# Autodesk Inventor assembly: Pok Mk3 Demo
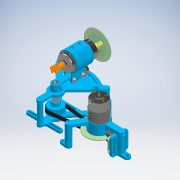
[picture p0: Inventor's stored thumbnail of the model, 180x180]
Saved by Autodesk Inventor 2018.2 (Build 222227000, 227)
## iProperties
Created: 2018-02-12
Part Number: Pok Mk3 Demo
Document SubType Name: Assembly
Designer: Moochster
Author: Moochster
## Documents named in this file (25)
- C:\Users\Moochster\OneDrive\Documents\2018 UBC\ELEC 391\Controller\cad\Pok Mk3 Demo.iam
- C:\Users\Moochster\OneDrive\Documents\2018 UBC\ELEC 391\Controller\cad\Rod 3-8in.ipt
- C:\Users\Moochster\OneDrive\Documents\2018 UBC\ELEC 391\Controller\cad\R1038_ZZ_W Bearing.ipt
- C:\Users\Moochster\OneDrive\Documents\2018 UBC\ELEC 391\Controller\cad\Yaw Platform Top.ipt
- C:\Users\Moochster\OneDrive\Documents\2018 UBC\ELEC 391\Controller\cad\Pok Header Mount.ipt
- C:\Users\Moochster\OneDrive\Documents\2018 UBC\ELEC 391\Controller\cad\JD5B-2655W-R.ipt
- C:\Users\Moochster\OneDrive\Documents\2018 UBC\ELEC 391\Controller\cad\Pok Default Pitch Motor Mount.ipt
- C:\Users\Moochster\OneDrive\Documents\2018 UBC\ELEC 391\Controller\cad\Laser Mount.ipt
- C:\Users\Moochster\Documents\Inventor\Content Center Files\R2018\en-US\AS 1110\AS 1110 - M3 x 20.ipt
- C:\Users\Moochster\Documents\Inventor\Content Center Files\R2018\en-US\AS 1112 (2)\AS 1112 - M3  Type 5.ipt
- C:\Users\Moochster\Documents\Inventor\Content Center Files\R2018\en-US\CNS 5050\CNS 5050 - A - 3.2 8.ipt
- C:\Users\Moochster\Documents\Inventor\Content Center Files\R2018\en-US\ANSI B18.3.1M(1)\ANSI B18.3.1M - M1.6x0.35 x 3(2).ipt
- C:\Users\Moochster\OneDrive\Documents\2018 UBC\ELEC 391\Controller\cad\Pok Mk3 Base.ipt
- C:\Users\Moochster\OneDrive\Documents\2018 UBC\ELEC 391\Controller\cad\Pok Mk3 Support.ipt
- C:\Users\Moochster\OneDrive\Documents\2018 UBC\ELEC 391\Controller\cad\Encoder Wheel (G16).ipt
- C:\Users\Moochster\OneDrive\Documents\2018 UBC\ELEC 391\Controller\cad\Shaft Encoder Adapter.ipt
- C:\Users\Moochster\OneDrive\Documents\2018 UBC\ELEC 391\Controller\cad\GP1A52HRJ00F (Large slot detector).ipt
- C:\Users\Moochster\OneDrive\Documents\2018 UBC\ELEC 391\Controller\cad\GT2 Gear Pinion.ipt
- C:\Users\Moochster\OneDrive\Documents\2018 UBC\ELEC 391\Controller\cad\GT2 Gear Big.ipt
- C:\Users\Moochster\OneDrive\Documents\2018 UBC\ELEC 391\Controller\cad\Pok Mk3 Yaw Motor Support.ipt
- C:\Users\Moochster\OneDrive\Documents\2018 UBC\ELEC 391\Controller\cad\Large Encoder PCB.ipt
- C:\Users\Moochster\OneDrive\Documents\2018 UBC\ELEC 391\Controller\cad\Nylon M3 4mm Spacer.ipt
- C:\Users\Moochster\OneDrive\Documents\2018 UBC\ELEC 391\Controller\cad\Pok Mk3 Yaw Motor Mount Mk2.ipt
- C:\Users\Moochster\OneDrive\Documents\2018 UBC\ELEC 391\Controller\cad\Pok Mk3 Yaw Motor Support Min.ipt
- C:\Users\Moochster\OneDrive\Documents\2018 UBC\ELEC 391\Controller\cad\Belt.ipt
## Components (41 placed, 24 different names)
1. Rod 3-8in:1 — Mate:1, Mate:2, Flush:1, Mate:10, Mate:23, Mate:24, Mate:42, Mate:70, Mate:71
2. R1038_ZZ_W Bearing:1 — Mate:1, Flush:1, Mate:60, Flush:17
3. R1038_ZZ_W Bearing:2 — Mate:2, Mate:5, Flush:2
4. Yaw Platform Top:1 — Mate:5, Flush:2, Mate:11, Angle:1, Insert:16
5. Pok Header Mount:1 — Mate:10, Mate:11, Mate:12, Flush:4, Mate:19, Mate:20, Mate:21, Angle:6, Mate:71
6. R1038_ZZ_W Bearing:3 — Mate:12, Flush:4
7. JD5B-2655W-R:1 — Mate:17, Mate:18, Mate:22, Flush:5, Angle:2, Tangent:1, Tangent:2, Mate:34, Mate:38, Angle:7
8. Laser Mount:1 — Mate:17, Mate:18
9. Pok Default Pitch Motor Mount:1 — Mate:19, Mate:20, Mate:21, Mate:22, Flush:5, Mate:25, Insert:1, Insert:3, Insert:5, Insert:7, Angle:2, Mate:26, Mate:27
10. AS 1110 - Metric M3 x 20:1 — Mate:25, Insert:2
11. AS 1110 - Metric M3 x 20:2 — Insert:6
12. CNS 5050 A - 3.2:4 — Insert:7, Insert:8
13. CNS 5050 A - 3.2:2 — Insert:5, Insert:6
14. CNS 5050 A - 3.2:3 — Insert:3, Insert:4
15. CNS 5050 A - 3.2:1 — Insert:1, Insert:2
16. AS 1112 (2) - Metric M3  Type 5:1 — Insert:8
17. AS 1112 (2) - Metric M3  Type 5:2 — Insert:4
18. Broached Socket Head Cap Screw - Metric M1.6x0.35 x 3:1 — Mate:26, Tangent:1
19. Broached Socket Head Cap Screw - Metric M1.6x0.35 x 3:2 — Mate:27, Tangent:2
20. Pok Mk3 Base:1 — Insert:13, Insert:14, Insert:15, Mate:60, Flush:17, Flush:18, Angle:5, Flush:20, Mate:68, Angle:7
21. Pok Mk3 Support:1 — Insert:13
22. Pok Mk3 Support:2 — Insert:15, Insert:16
23. Pok Mk3 Support:3 — Insert:14
24. JD5B-2655W-R:2 — Mate:32, Mate:41, Mate:44, Mate:53, Mate:55
25. Encoder Wheel (G16):1 — Mate:32, Mate:43, Mate:44, Mate:69
26. Encoder Wheel (G16):2 — Mate:35, Mate:36, Mate:37
27. Shaft Encoder Adapter:1 — Mate:34, Mate:35, Mate:36, Mate:37, Mate:38
28. GP1A52HRJ00F (Large slot detector):3 — Mate:50, Flush:13, Flush:14, Mate:51, Flush:15
29. GP1A52HRJ00F (Large slot detector):4 — Mate:50, Flush:13, Flush:14, Flush:16
30. GT2 Gear Pinion:1 — Mate:41, Mate:43, Flush:10, Mate:67, Mate:69, Rotation:1
31. GT2 Gear Big:1 — Mate:42, Flush:10, Angle:6, Mate:65, Mate:66, Rotation:1, Mate:70
32. Pok Mk3 Yaw Motor Support:4 — Mate:52, Mate:54, Angle:4, Tangent:3, Tangent:4, Mate:62
33. Large Encoder PCB:1 — Mate:51, Flush:15, Flush:16, Mate:52, Insert:9, Insert:10, Insert:11, Insert:12
34. Nylon M3 4mm Spacer:1 — Insert:10, Tangent:4
35. Nylon M3 4mm Spacer:2 — Insert:9
36. Nylon M3 4mm Spacer:3 — Insert:12
37. Nylon M3 4mm Spacer:4 — Insert:11, Tangent:3
38. Pok Mk3 Yaw Motor Mount Mk2:1 — Mate:53, Mate:54, Angle:4, Mate:55, Mate:56, Mate:57, Mate:58, Mate:59, Angle:5, Mate:62, Mate:68
39. Pok Mk3 Yaw Motor Support Min:1 — Mate:56, Mate:58, Mate:64
40. Pok Mk3 Yaw Motor Support Min:2 — Mate:57, Mate:59, Flush:18, Mate:63
41. Belt:1 — Mate:65, Mate:66, Mate:67
## Relationships (87: Mate 48, Insert 16, Flush 12, Angle 6, Tangent 4, RelateRotation 1)
- Mate:1: Rod 3-8in:1 ↔ R1038_ZZ_W Bearing:1
- Mate:2: Rod 3-8in:1 ↔ R1038_ZZ_W Bearing:2
- Flush:1: Rod 3-8in:1 ↔ R1038_ZZ_W Bearing:1
- Mate:5: R1038_ZZ_W Bearing:2 ↔ Yaw Platform Top:1
- Flush:2: R1038_ZZ_W Bearing:2 ↔ Yaw Platform Top:1
- Mate:10: Rod 3-8in:1 ↔ Pok Header Mount:1
- Mate:11 (0.2 mm): Yaw Platform Top:1 ↔ Pok Header Mount:1
- Mate:12: Pok Header Mount:1 ↔ R1038_ZZ_W Bearing:3
- Flush:4 (1 mm): Pok Header Mount:1 ↔ R1038_ZZ_W Bearing:3
- Mate:17: JD5B-2655W-R:1 ↔ Laser Mount:1
- Mate:18 (1 mm): JD5B-2655W-R:1 ↔ Laser Mount:1
- Mate:19: Pok Header Mount:1 ↔ Pok Default Pitch Motor Mount:1
- Mate:20: Pok Header Mount:1 ↔ Pok Default Pitch Motor Mount:1
- Mate:21 (0.1 mm): Pok Header Mount:1 ↔ Pok Default Pitch Motor Mount:1
- Mate:22: JD5B-2655W-R:1 ↔ Pok Default Pitch Motor Mount:1
- Mate:23: Rod 3-8in:1
- Mate:24: Rod 3-8in:1
- Angle:1 (0 deg): Yaw Platform Top:1
- Flush:5 (-10 mm): JD5B-2655W-R:1 ↔ Pok Default Pitch Motor Mount:1
- Mate:25: Pok Default Pitch Motor Mount:1 ↔ AS 1110 - Metric M3 x 20:1
- Insert:1: Pok Default Pitch Motor Mount:1 ↔ CNS 5050 A - 3.2:1
- Insert:2: AS 1110 - Metric M3 x 20:1 ↔ CNS 5050 A - 3.2:1
- Insert:3: Pok Default Pitch Motor Mount:1 ↔ CNS 5050 A - 3.2:3
- Insert:4: CNS 5050 A - 3.2:3 ↔ AS 1112 (2) - Metric M3  Type 5:2
- Insert:5: Pok Default Pitch Motor Mount:1 ↔ CNS 5050 A - 3.2:2
- Insert:6: AS 1110 - Metric M3 x 20:2 ↔ CNS 5050 A - 3.2:2
- Insert:7: Pok Default Pitch Motor Mount:1 ↔ CNS 5050 A - 3.2:4
- Insert:8: CNS 5050 A - 3.2:4 ↔ AS 1112 (2) - Metric M3  Type 5:1
- Angle:2 (180 deg): JD5B-2655W-R:1 ↔ Pok Default Pitch Motor Mount:1
- Mate:26: Pok Default Pitch Motor Mount:1 ↔ Broached Socket Head Cap Screw - Metric M1.6x0.35 x 3:1
- Tangent:1: JD5B-2655W-R:1 ↔ Broached Socket Head Cap Screw - Metric M1.6x0.35 x 3:1
- Mate:27: Pok Default Pitch Motor Mount:1 ↔ Broached Socket Head Cap Screw - Metric M1.6x0.35 x 3:2
- Tangent:2: JD5B-2655W-R:1 ↔ Broached Socket Head Cap Screw - Metric M1.6x0.35 x 3:2
- Mate:32: JD5B-2655W-R:2 ↔ Encoder Wheel (G16):1
- Mate:34: JD5B-2655W-R:1 ↔ Shaft Encoder Adapter:1
- Mate:35: Encoder Wheel (G16):2 ↔ Shaft Encoder Adapter:1
- Mate:36: Encoder Wheel (G16):2 ↔ Shaft Encoder Adapter:1
- Mate:37: Encoder Wheel (G16):2 ↔ Shaft Encoder Adapter:1
- Mate:38 (0.25 mm): JD5B-2655W-R:1 ↔ Shaft Encoder Adapter:1
- Mate:41: JD5B-2655W-R:2 ↔ GT2 Gear Pinion:1
- Mate:42: Rod 3-8in:1 ↔ GT2 Gear Big:1
- Mate:43: Encoder Wheel (G16):1 ↔ GT2 Gear Pinion:1
- Mate:44 (0.5 mm): JD5B-2655W-R:2 ↔ Encoder Wheel (G16):1
- Flush:10: GT2 Gear Pinion:1 ↔ GT2 Gear Big:1
- Mate:50 (0.7 mm): GP1A52HRJ00F (Large slot detector):3 ↔ GP1A52HRJ00F (Large slot detector):4
- Flush:13: GP1A52HRJ00F (Large slot detector):3 ↔ GP1A52HRJ00F (Large slot detector):4
- Flush:14: GP1A52HRJ00F (Large slot detector):3 ↔ GP1A52HRJ00F (Large slot detector):4
- Mate:51 (0.1 mm): GP1A52HRJ00F (Large slot detector):3 ↔ Large Encoder PCB:1
- Flush:15 (2 mm): GP1A52HRJ00F (Large slot detector):3 ↔ Large Encoder PCB:1
- Flush:16 (7 mm): GP1A52HRJ00F (Large slot detector):4 ↔ Large Encoder PCB:1
- Mate:52 (4 mm): Pok Mk3 Yaw Motor Support:4 ↔ Large Encoder PCB:1
- Mate:53: JD5B-2655W-R:2 ↔ Pok Mk3 Yaw Motor Mount Mk2:1
- Mate:54: Pok Mk3 Yaw Motor Support:4 ↔ Pok Mk3 Yaw Motor Mount Mk2:1
- Angle:4 (0 deg): Pok Mk3 Yaw Motor Support:4 ↔ Pok Mk3 Yaw Motor Mount Mk2:1
- Mate:55: JD5B-2655W-R:2 ↔ Pok Mk3 Yaw Motor Mount Mk2:1
- Mate:56: Pok Mk3 Yaw Motor Mount Mk2:1 ↔ Pok Mk3 Yaw Motor Support Min:1
- Mate:57: Pok Mk3 Yaw Motor Mount Mk2:1 ↔ Pok Mk3 Yaw Motor Support Min:2
- Mate:58 (0.1 mm): Pok Mk3 Yaw Motor Mount Mk2:1 ↔ Pok Mk3 Yaw Motor Support Min:1
- Mate:59 (0.1 mm): Pok Mk3 Yaw Motor Mount Mk2:1 ↔ Pok Mk3 Yaw Motor Support Min:2
- Insert:9: Large Encoder PCB:1 ↔ Nylon M3 4mm Spacer:2
- Insert:10: Large Encoder PCB:1 ↔ Nylon M3 4mm Spacer:1
- Insert:11: Large Encoder PCB:1 ↔ Nylon M3 4mm Spacer:4
- Insert:12: Large Encoder PCB:1 ↔ Nylon M3 4mm Spacer:3
- Tangent:3: Pok Mk3 Yaw Motor Support:4 ↔ Nylon M3 4mm Spacer:4
- Tangent:4: Pok Mk3 Yaw Motor Support:4 ↔ Nylon M3 4mm Spacer:1
- Insert:13 (0.1 mm): Pok Mk3 Base:1 ↔ Pok Mk3 Support:1
- Insert:14 (0.1 mm): Pok Mk3 Base:1 ↔ Pok Mk3 Support:3
- Insert:15 (0.1 mm): Pok Mk3 Base:1 ↔ Pok Mk3 Support:2
- Mate:60: R1038_ZZ_W Bearing:1 ↔ Pok Mk3 Base:1
- Insert:16 (0.1 mm): Yaw Platform Top:1 ↔ Pok Mk3 Support:2
- Flush:17: R1038_ZZ_W Bearing:1 ↔ Pok Mk3 Base:1
- Flush:18: Pok Mk3 Base:1 ↔ Pok Mk3 Yaw Motor Support Min:2
- Angle:5 (0 deg): Pok Mk3 Base:1 ↔ Pok Mk3 Yaw Motor Mount Mk2:1
- Angle:6 (0 deg): Pok Header Mount:1 ↔ GT2 Gear Big:1
- Mate:62 (0.1 mm): Pok Mk3 Yaw Motor Support:4 ↔ Pok Mk3 Yaw Motor Mount Mk2:1
- Flush:20 (-48 mm): Pok Mk3 Base:1
- Mate:63: Pok Mk3 Yaw Motor Support Min:2
- Mate:64: Pok Mk3 Yaw Motor Support Min:1
- Mate:65: GT2 Gear Big:1 ↔ Belt:1
- Mate:66 (0.2 mm): GT2 Gear Big:1 ↔ Belt:1
- Mate:67: GT2 Gear Pinion:1 ↔ Belt:1
- Mate:68: Pok Mk3 Base:1 ↔ Pok Mk3 Yaw Motor Mount Mk2:1
- Mate:69: Encoder Wheel (G16):1 ↔ GT2 Gear Pinion:1
- Rotation:1 [RelateRotation] (3.5 ul): GT2 Gear Pinion:1 ↔ GT2 Gear Big:1
- Mate:70: Rod 3-8in:1 ↔ GT2 Gear Big:1
- Mate:71: Rod 3-8in:1 ↔ Pok Header Mount:1
- Angle:7 (0 deg): JD5B-2655W-R:1 ↔ Pok Mk3 Base:1
